# Autodesk Inventor assembly: Deck_Bushing
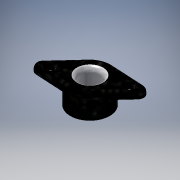
[picture p0: Inventor's stored thumbnail of the model, 180x180]
Saved by Autodesk Inventor 2016 (Build 200138000, 138)
## iProperties
Created: 2016-05-07
Part Number: Deck_Bushing
Document SubType Name: Assembly
Designer: agmle
Mass: 5.07542 g
Surface Area: 18.6321 cm^2
Volume: 1.65164 cm^3
Density: 3.07295 g/cm^3
Author: agmle
## Documents named in this file (3)
- C:\Users\agmle\BitTorrent Sync\private\projects\Creekfleet_Timer\hardware\CAD\Remote\Deck_Bushing.iam
- C:\Users\agmle\BitTorrent Sync\private\projects\Creekfleet_Timer\hardware\CAD\Remote\Deck_Bushing_Liner.ipt
- C:\Users\agmle\BitTorrent Sync\private\projects\Creekfleet_Timer\hardware\CAD\Remote\Deck_Bushing_Outer.ipt
## Components (2 placed, 2 different names)
1. Deck_Bushing_Liner:1 — Insert:1
2. Deck_Bushing_Outer:1 — Insert:1
## Relationships (1: Insert 1)
- Insert:1: Deck_Bushing_Liner:1 ↔ Deck_Bushing_Outer:1
